# Autodesk Inventor assembly: DIL16-Socket+Package
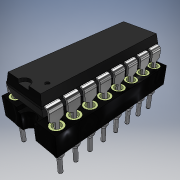
[picture p0: Inventor's stored thumbnail of the model, 180x180]
Saved by Autodesk Inventor 2018 (Build 220112000, 112)
## iProperties
Created: 2020-04-20
Part Number: DIL16-Socket+Package
Material: Všeobecné
Document SubType Name: Assembly
Designer: Jozko Mrkvicka
Author: Jozko Mrkvicka
## Documents named in this file (3)
- F:\Workspace\Projekty\Library\DIL16-Socket+Package.iam
- F:\Workspace\Projekty\Library\DIL16-Socket.ipt
- F:\Workspace\Projekty\Library\DIL16-Package.ipt
## Components (2 placed, 2 different names)
1. DIL16-Socket:1 — Vložit:1, Proti sobě:1
2. DIL16-Package:1 — Vložit:1, Proti sobě:1
## Relationships (2: Insert 1, Mate 1)
- Vložit:1 [Insert]: DIL16-Socket:1 ↔ DIL16-Package:1
- Proti sobě:1 [Mate]: DIL16-Socket:1 ↔ DIL16-Package:1
